# Autodesk Inventor assembly: Assembly2
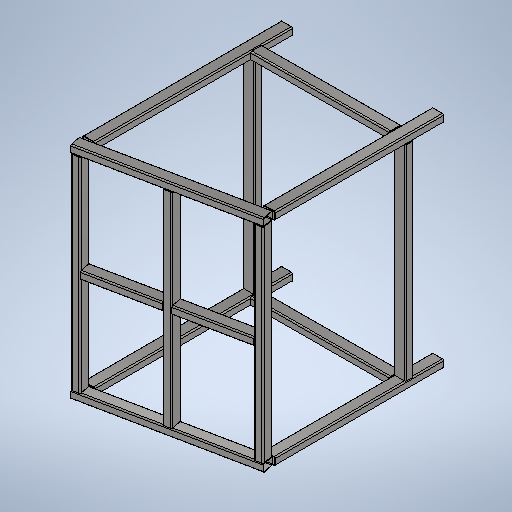
[picture p0: Inventor's stored thumbnail of the model, 512x512]
Saved by Autodesk Inventor 2025 (Build 290162010, 162A)
## iProperties
Created: 2024-09-20
Part Number: Assembly2
Document SubType Name: Assembly
Designer: admin
Author: admin
## Documents named in this file (5)
- C:\Users\admin\YandexDisk-badmisterfox\домашниий пк\Inventor\BSH_Beshkino_bio_tank\Assembly2.iam
- C:\Users\admin\YandexDisk-badmisterfox\домашниий пк\Inventor\BSH_Beshkino_bio_tank\Тумба 1.iam
- C:\Users\admin\YandexDisk-badmisterfox\домашниий пк\Inventor\BSH_Beshkino_bio_tank\Ноги тумба 2.iam
- C:\Users\admin\YandexDisk-badmisterfox\домашниий пк\Inventor\BSH_Beshkino_bio_tank\Ноги тумба 1.iam
- C:\Users\admin\YandexDisk-badmisterfox\домашниий пк\Inventor\BSH_Beshkino_bio_tank\ISO 4019 - 60x40x3 - 691.ipt
## Components (5 placed, 4 different names)
1. Тумба 1:1 [sub-assembly]
2. Ноги тумба 2:1 [sub-assembly]
3. Ноги тумба 1:1 [sub-assembly]
4. ISO 4019 - 60x40x3 - 691:1
5. ISO 4019 - 60x40x3 - 691:2
## Relationships (13: Flush 7, Mate 6)
- [Flush]: Ноги тумба 2:1 ↔ Ноги тумба 1:1
- [Mate] (691 mm): Ноги тумба 2:1 ↔ Ноги тумба 1:1
- [Mate]: Ноги тумба 1:1 ↔ ISO 4019 - 60x40x3 - 691:1
- [Flush] (150 mm): Ноги тумба 1:1 ↔ ISO 4019 - 60x40x3 - 691:1
- [Flush]: Ноги тумба 1:1 ↔ ISO 4019 - 60x40x3 - 691:1
- [Mate]: Ноги тумба 1:1 ↔ ISO 4019 - 60x40x3 - 691:2
- [Flush]: Ноги тумба 1:1 ↔ ISO 4019 - 60x40x3 - 691:2
- [Flush] (150 mm): Ноги тумба 1:1 ↔ ISO 4019 - 60x40x3 - 691:2
- [Flush]: Ноги тумба 2:1 ↔ Ноги тумба 1:1
- [Flush]: Тумба 1:1 ↔ Ноги тумба 2:1
- [Mate]: Тумба 1:1 ↔ Ноги тумба 1:1
- [Mate]: Тумба 1:1 ↔ Ноги тумба 1:1
- [Mate]: Тумба 1:1 ↔ Ноги тумба 2:1
